# Autodesk Inventor assembly: New Pin
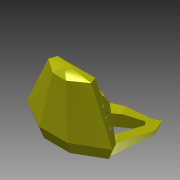
[picture p0: Inventor's stored thumbnail of the model, 180x180]
Saved by Autodesk Inventor 2014 (Build 180170000, 170)
## iProperties
Created: 2015-01-24
Part Number: New Pin
Document SubType Name: Assembly
Designer: Spooner
Author: Spooner
## Documents named in this file (3)
- C:\Users\Spooner\Documents\Inventor\RoboCat Gen 2\New Pin.iam
- C:\Users\Spooner\Documents\Inventor\RoboCat Gen 2\Disk.ipt
- C:\Users\Spooner\Documents\Inventor\RoboCat Gen 2\Cat.ipt
## Components (2 placed, 2 different names)
1. Disk:1 — Angle:1, Tangent:1, Mate:1, Mate:2, Mate:3
2. Cat:1 — Angle:1, Tangent:1, Mate:1, Angle:2
## Relationships (6: Mate 3, Angle 2, Tangent 1)
- Angle:1 (180 deg): Disk:1 ↔ Cat:1
- Tangent:1: Disk:1 ↔ Cat:1
- Mate:1: Disk:1 ↔ Cat:1
- Mate:2: Disk:1
- Mate:3: Disk:1
- Angle:2 (-90 deg): Cat:1
